# Autodesk Inventor assembly: HipJoint
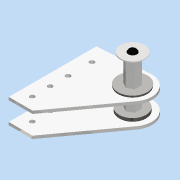
[picture p0: Inventor's stored thumbnail of the model, 180x180]
Saved by Autodesk Inventor 2022 (Build 260153000, 153)
## iProperties
Created: 2023-02-11
Part Number: HipJoint
Document SubType Name: Assembly
Designer: coled
Author: coled
## Documents named in this file (6)
- D:\Behrend\RoboticsClub\New folder\HipJoint.iam
- D:\Behrend\RoboticsClub\New folder\Bearing.ipt
- D:\Behrend\RoboticsClub\New folder\Bracket.ipt
- D:\Behrend\RoboticsClub\New folder\HexShaft.ipt
- D:\Behrend\RoboticsClub\New folder\Washer.ipt
- D:\Behrend\RoboticsClub\New folder\Screw.ipt
## Components (9 placed, 5 different names)
1. Bearing:1 — Mate:1, Mate:2, Mate:4
2. Bracket:1 — Mate:1, Mate:2, Mate:3
3. Bracket:2 — Mate:3, Mate:4, Mate:5, Mate:6
4. Bearing:2 — Mate:5, Mate:6, Mate:7, Flush:1, Mate:8
5. HexShaft:1 — Mate:7, Flush:1, Mate:9, Mate:10, Mate:11, Mate:16
6. Washer:1 — Mate:10, Mate:11, Mate:14, Mate:15
7. Washer:2 — Mate:8, Mate:9, Mate:12
8. Screw:1 — Mate:14, Mate:15
9. Screw:2 — Mate:12, Mate:16
## Relationships (16: Mate 15, Flush 1)
- Mate:1: Bearing:1 ↔ Bracket:1
- Mate:2: Bearing:1 ↔ Bracket:1
- Mate:3 (20 mm): Bracket:1 ↔ Bracket:2
- Mate:4: Bearing:1 ↔ Bracket:2
- Mate:5: Bracket:2 ↔ Bearing:2
- Mate:6: Bracket:2 ↔ Bearing:2
- Mate:7: Bearing:2 ↔ HexShaft:1
- Flush:1: Bearing:2 ↔ HexShaft:1
- Mate:8: Bearing:2 ↔ Washer:2
- Mate:9: HexShaft:1 ↔ Washer:2
- Mate:10: HexShaft:1 ↔ Washer:1
- Mate:11: HexShaft:1 ↔ Washer:1
- Mate:12: Washer:2 ↔ Screw:2
- Mate:14: Washer:1 ↔ Screw:1
- Mate:15: Washer:1 ↔ Screw:1
- Mate:16: HexShaft:1 ↔ Screw:2
